# Autodesk Inventor assembly: SAFRS-A-0014
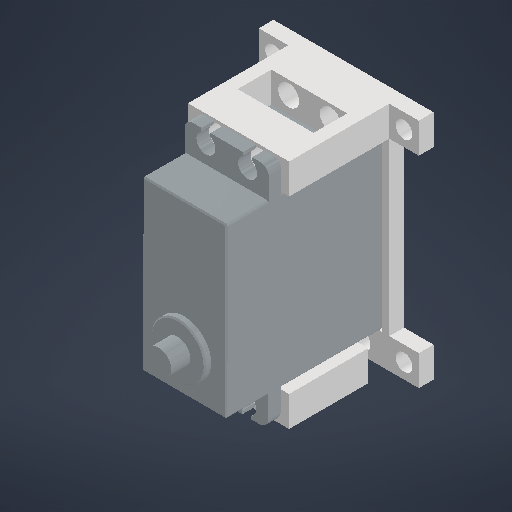
[picture p0: Inventor's stored thumbnail of the model, 512x512]
Saved by Autodesk Inventor 2026.2 (Build 302298000, 298)
## iProperties
Created: 2025-11-24
Part Number: SAFRS-A-0014
Document SubType Name: Assembly
Designer: jaewook
Author: jaewook
Title: Yaw Motor Mount Assembly
## Documents named in this file (3)
- C:\Users\jk000\OneDrive\Desktop\git\SAFRS\mechanical\inventor\02__subassemblies\yaw_motor_mount.iam
- C:\Users\jk000\OneDrive\Desktop\git\SAFRS\mechanical\inventor\01_parts\yaw_motor_mount.ipt
- C:\Users\jk000\OneDrive\Desktop\git\SAFRS\mechanical\inventor\01_parts\servo_ds35mg_180.ipt
## Components (2 placed, 2 different names)
1. yaw_motor_mount:1 — 메이트:1
2. servo_ds35mg_180:1 — 메이트:1
## Relationships (1: Mate 1)
- 메이트:1 [Mate]: yaw_motor_mount:1 ↔ servo_ds35mg_180:1
